# Autodesk Inventor assembly: Electromanetic brake
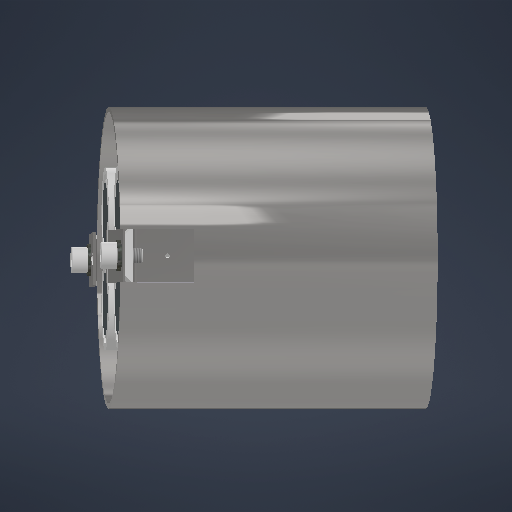
[picture p0: Inventor's stored thumbnail of the model, 512x512]
Saved by Autodesk Inventor 2026.3 (Build 303398000, 398)
## iProperties
Created: 2026-08-09
Part Number: Electromanetic brake
Document SubType Name: Weldment
Designer: matot
Weld Material: Aluminum 6061, Welded
Author: matot
## Documents named in this file (5)
- C:\Users\matot\OneDrive - Stellenbosch University\2026\MechatronicsProject478\Building the joint\Joint Assembly\Electromanetic brake.iam
- C:\Users\matot\OneDrive - Stellenbosch University\2026\MechatronicsProject478\Building the joint\Joint Assembly\Electromagnet final_key.iam
- C:\Users\matot\OneDrive - Stellenbosch University\2026\MechatronicsProject478\Building the joint\Joint Assembly\Pressure platform.ipt
- C:\Users\matot\OneDrive - Stellenbosch University\Documents\Inventor\Content Center Files\R2026\en-US\ISO 7091\ISO 7091 - ST 6 - 100 HV.ipt
- C:\Users\matot\OneDrive - Stellenbosch University\2026\MechatronicsProject478\Building the joint\Joint Assembly\din_912-m6x1-10-10_9.ipt
## Components (7 placed, 4 different names)
1. Electromagnet final_key:1 [sub-assembly] — Insert:5, Flush:1, Flush:2, Insert:6, Flush:3
2. Pressure platform:1 — Insert:6, Flush:3, Insert:7
3. Pressure platform:2 — Insert:5, Flush:1, Flush:2, Insert:8
4. ISO 7091 ST 6 - 100 HV:1 — Insert:7, Insert:9
5. ISO 7091 ST 6 - 100 HV:2 — Insert:8, Insert:10
6. din_912-m6x1-10-10_9:1 — Insert:9
7. din_912-m6x1-10-10_9:2 — Insert:10
## Relationships (9: Insert 6, Flush 3)
- Insert:5: Electromagnet final_key:1 ↔ Pressure platform:2
- Flush:1: Electromagnet final_key:1 ↔ Pressure platform:2
- Flush:2: Electromagnet final_key:1 ↔ Pressure platform:2
- Insert:6: Electromagnet final_key:1 ↔ Pressure platform:1
- Flush:3: Electromagnet final_key:1 ↔ Pressure platform:1
- Insert:7: Pressure platform:1 ↔ ISO 7091 ST 6 - 100 HV:1
- Insert:8: Pressure platform:2 ↔ ISO 7091 ST 6 - 100 HV:2
- Insert:9: ISO 7091 ST 6 - 100 HV:1 ↔ din_912-m6x1-10-10_9:1
- Insert:10: ISO 7091 ST 6 - 100 HV:2 ↔ din_912-m6x1-10-10_9:2
